# Autodesk Inventor assembly: Assembly1
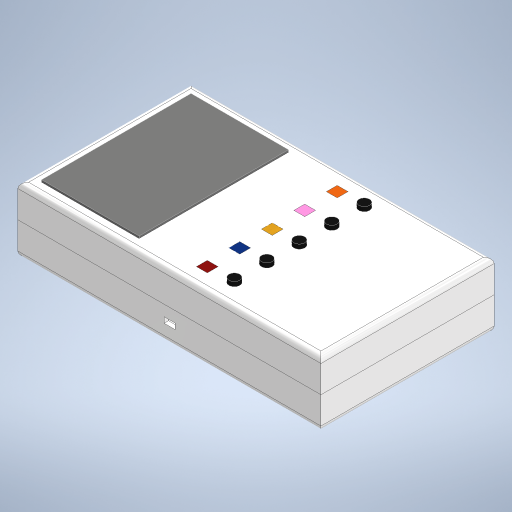
[picture p0: Inventor's stored thumbnail of the model, 512x512]
Saved by Autodesk Inventor 2023 (Build 270158000, 158)
## iProperties
Created: 2022-11-17
Part Number: Assembly1
Document SubType Name: Assembly
Designer: spfow
Author: spfow
## Documents named in this file (8)
- C:\Users\spfow\OneDrive\Documents\ECE_414\Final_Project\CAD\Assembly1.iam
- C:\Users\spfow\OneDrive\Documents\ECE_414\Final_Project\CAD\Battery Cover.ipt
- C:\Users\spfow\OneDrive\Documents\ECE_414\Final_Project\CAD\CaseTop.ipt
- C:\Users\spfow\OneDrive\Documents\ECE_414\Final_Project\CAD\CaseBottom.ipt
- C:\Users\spfow\OneDrive\Documents\ECE_414\Final_Project\CAD\button.ipt
- C:\Users\spfow\OneDrive\Documents\ECE_414\Final_Project\CAD\LCD.ipt
- C:\Users\spfow\OneDrive\Documents\ECE_414\Final_Project\CAD\LED.ipt
- C:\Users\spfow\OneDrive\Documents\ECE_414\Final_Project\CAD\Speaker.ipt
## Components (16 placed, 7 different names)
1. Battery Cover:1 — Mate:19, Mate:20, Mate:21
2. CaseTop:1 — Insert:1, Insert:2, Insert:3, Insert:4, Insert:5, Mate:1, Mate:2, Mate:3, Mate:4, Mate:5, Mate:6, Mate:7, Mate:8, Mate:9, Mate:10, Mate:11, Mate:12, Mate:13, Mate:14, Mate:15, Mate:16, Mate:17, Mate:18, Mate:22, Flush:1, Flush:2
3. CaseBottom:1 — Insert:6, Insert:7, Mate:19, Mate:20, Mate:21, Mate:22, Flush:1, Flush:2
4. button:1 — Insert:1
5. button:2 — Insert:2
6. button:3 — Insert:3
7. button:4 — Insert:4
8. button:5 — Insert:5
9. LCD:1 — Mate:1, Mate:2, Mate:3
10. LED:1 — Mate:4, Mate:9, Mate:14
11. LED:2 — Mate:5, Mate:11, Mate:16
12. LED:3 — Mate:6, Mate:10, Mate:15
13. LED:4 — Mate:7, Mate:12, Mate:17
14. LED:5 — Mate:8, Mate:13, Mate:18
15. Speaker:1 — Insert:6
16. Speaker:2 — Insert:7
## Relationships (31: Mate 22, Insert 7, Flush 2)
- Insert:1: CaseTop:1 ↔ button:1
- Insert:2: CaseTop:1 ↔ button:2
- Insert:3: CaseTop:1 ↔ button:3
- Insert:4: CaseTop:1 ↔ button:4
- Insert:5: CaseTop:1 ↔ button:5
- Mate:1: CaseTop:1 ↔ LCD:1
- Mate:2: CaseTop:1 ↔ LCD:1
- Mate:3: CaseTop:1 ↔ LCD:1
- Mate:4: CaseTop:1 ↔ LED:1
- Mate:5: CaseTop:1 ↔ LED:2
- Mate:6: CaseTop:1 ↔ LED:3
- Mate:7: CaseTop:1 ↔ LED:4
- Mate:8: CaseTop:1 ↔ LED:5
- Mate:9: CaseTop:1 ↔ LED:1
- Mate:10: CaseTop:1 ↔ LED:3
- Mate:11: CaseTop:1 ↔ LED:2
- Mate:12: CaseTop:1 ↔ LED:4
- Mate:13: CaseTop:1 ↔ LED:5
- Mate:14: CaseTop:1 ↔ LED:1
- Mate:15: CaseTop:1 ↔ LED:3
- Mate:16: CaseTop:1 ↔ LED:2
- Mate:17: CaseTop:1 ↔ LED:4
- Mate:18: CaseTop:1 ↔ LED:5
- Insert:6: CaseBottom:1 ↔ Speaker:1
- Insert:7: CaseBottom:1 ↔ Speaker:2
- Mate:19: Battery Cover:1 ↔ CaseBottom:1
- Mate:20: Battery Cover:1 ↔ CaseBottom:1
- Mate:21 (0.254 mm): Battery Cover:1 ↔ CaseBottom:1
- Mate:22: CaseTop:1 ↔ CaseBottom:1
- Flush:1: CaseTop:1 ↔ CaseBottom:1
- Flush:2: CaseTop:1 ↔ CaseBottom:1
